# Autodesk Inventor assembly: SuperCleaner
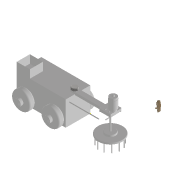
[picture p0: Inventor's stored thumbnail of the model, 180x180]
Saved by Autodesk Inventor 2022 (Build 260153000, 153)
## iProperties
Created: 2021-06-23
Part Number: SuperCleaner
Document SubType Name: Assembly
Designer: LENOVO
Author: LENOVO
## Documents named in this file (7)
- C:\Users\LENOVO\Documents\Inventor\explo\SuperCleaner.iam
- C:\Users\LENOVO\Documents\Inventor\explo\bodycar.ipt
- C:\Users\LENOVO\Documents\Inventor\explo\axle.ipt
- C:\Users\LENOVO\Documents\Inventor\explo\wheel.ipt
- C:\Users\LENOVO\Documents\Inventor\explo\Assembly3.iam
- C:\Users\LENOVO\Documents\Inventor\explo\part1.ipt
- C:\Users\LENOVO\Downloads\HUMAN HAND.ipt
## Components (12 placed, 6 different names)
1. bodycar:1 — Mate:1, Mate:2, Mate:5, Mate:6, Mate:9, Mate:10, Mate:14, Mate:15, Mate:18, Mate:19, Mate:20, Mate:21
2. axle:1 — Mate:3, Mate:4
3. axle:2 — Mate:7, Mate:8
4. axle:3 — Mate:12, Mate:13
5. axle:4 — Mate:11, Mate:16, Mate:17
6. wheel:1 — Mate:1, Mate:2, Mate:3, Mate:4
7. wheel:2 — Mate:5, Mate:6, Mate:7, Mate:8
8. wheel:3 — Mate:9, Mate:10, Mate:11, Mate:12, Mate:13
9. wheel:4 — Mate:14, Mate:15, Mate:16, Mate:17
10. Assembly3:1 [sub-assembly] — Mate:18, Mate:19
11. part1:1 — Mate:20, Mate:21
12. HUMAN HAND:1
## Relationships (21: Mate 21)
- Mate:1: bodycar:1 ↔ wheel:1
- Mate:2: bodycar:1 ↔ wheel:1
- Mate:3: axle:1 ↔ wheel:1
- Mate:4: axle:1 ↔ wheel:1
- Mate:5: bodycar:1 ↔ wheel:2
- Mate:6: bodycar:1 ↔ wheel:2
- Mate:7: axle:2 ↔ wheel:2
- Mate:8: axle:2 ↔ wheel:2
- Mate:9: bodycar:1 ↔ wheel:3
- Mate:10: bodycar:1 ↔ wheel:3
- Mate:11: axle:4 ↔ wheel:3
- Mate:12: axle:3 ↔ wheel:3
- Mate:13: axle:3 ↔ wheel:3
- Mate:14: bodycar:1 ↔ wheel:4
- Mate:15: bodycar:1 ↔ wheel:4
- Mate:16: axle:4 ↔ wheel:4
- Mate:17: axle:4 ↔ wheel:4
- Mate:18: bodycar:1 ↔ Assembly3:1
- Mate:19: bodycar:1 ↔ Assembly3:1
- Mate:20: bodycar:1 ↔ part1:1
- Mate:21: bodycar:1 ↔ part1:1
